# Autodesk Inventor assembly: POM_T5_16
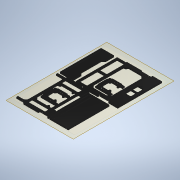
[picture p0: Inventor's stored thumbnail of the model, 180x180]
Saved by Autodesk Inventor 2020 (Build 240168000, 168)
## iProperties
Created: 2021-08-27
Part Number: POM_T5_16
Document SubType Name: Assembly
Designer: Masato
Author: Masato
## Documents named in this file (8)
- C:\Inventor\SUSTAINA-OP\Cam\POM_T5_16.iam
- C:\Inventor\SUSTAINA-OP\Cam\DisposableBoard.ipt
- C:\Inventor\SUSTAINA-OP\UpperBody\Cockpit\Cockpit_front_frame.ipt
- C:\Inventor\SUSTAINA-OP\UpperBody\Cockpit\Cockpit_carrier_board_frame.ipt
- C:\Inventor\SUSTAINA-OP\UpperBody\Cockpit\Cockpit_circuit_board_frame.ipt
- C:\Inventor\SUSTAINA-OP\UpperBody\Cockpit\Cockpit_battery_back_door.ipt
- C:\Inventor\SUSTAINA-OP\UpperBody\Cockpit\Cockpit_top_frame.ipt
- C:\Inventor\SUSTAINA-OP\UpperBody\Head\Camera_root_frame_e-CAM50_CUNX.ipt
## Components (8 placed, 7 different names)
1. DisposableBoard:1 — メイト:2, メイト:1, フラッシュ:1, フラッシュ:2, メイト:4, メイト:5, メイト:6, メイト:7, フラッシュ:3, フラッシュ:4, メイト:13, メイト:14, メイト:15
2. Cockpit_front_frame:1 — メイト:4, フラッシュ:5, メイト:9
3. Cockpit_carrier_board_frame:1 — メイト:5, フラッシュ:3, フラッシュ:4, フラッシュ:5, フラッシュ:6, メイト:8, メイト:9, メイト:10, メイト:11, メイト:16, メイト:17
4. Cockpit_circuit_board_frame:1 — メイト:7, メイト:10, メイト:11, メイト:12, フラッシュ:7, メイト:18, メイト:19
5. Cockpit_battery_back_door:1 — メイト:6, フラッシュ:6, メイト:8
6. Cockpit_top_frame:1 — メイト:12, メイト:13, フラッシュ:7
7. Camera_root_frame_e-CAM50_CUNX:1 — メイト:14, メイト:16, メイト:17
8. Camera_root_frame_e-CAM50_CUNX:2 — メイト:15, メイト:18, メイト:19
## Relationships (25: Mate 18, Flush 7)
- メイト:2 [Mate]: DisposableBoard:1
- メイト:1 [Mate]: DisposableBoard:1
- フラッシュ:1 [Flush]: DisposableBoard:1
- フラッシュ:2 [Flush]: DisposableBoard:1
- メイト:4 [Mate]: DisposableBoard:1 ↔ Cockpit_front_frame:1
- メイト:5 [Mate]: DisposableBoard:1 ↔ Cockpit_carrier_board_frame:1
- メイト:6 [Mate]: DisposableBoard:1 ↔ Cockpit_battery_back_door:1
- メイト:7 [Mate]: DisposableBoard:1 ↔ Cockpit_circuit_board_frame:1
- フラッシュ:3 [Flush] (2 mm): DisposableBoard:1 ↔ Cockpit_carrier_board_frame:1
- フラッシュ:4 [Flush] (2 mm): DisposableBoard:1 ↔ Cockpit_carrier_board_frame:1
- フラッシュ:5 [Flush]: Cockpit_front_frame:1 ↔ Cockpit_carrier_board_frame:1
- フラッシュ:6 [Flush]: Cockpit_carrier_board_frame:1 ↔ Cockpit_battery_back_door:1
- メイト:8 [Mate] (2.5 mm): Cockpit_carrier_board_frame:1 ↔ Cockpit_battery_back_door:1
- メイト:9 [Mate] (2.5 mm): Cockpit_front_frame:1 ↔ Cockpit_carrier_board_frame:1
- メイト:10 [Mate] (2.5 mm): Cockpit_carrier_board_frame:1 ↔ Cockpit_circuit_board_frame:1
- メイト:11 [Mate] (2.5 mm): Cockpit_carrier_board_frame:1 ↔ Cockpit_circuit_board_frame:1
- メイト:12 [Mate] (2.5 mm): Cockpit_circuit_board_frame:1 ↔ Cockpit_top_frame:1
- メイト:13 [Mate]: DisposableBoard:1 ↔ Cockpit_top_frame:1
- フラッシュ:7 [Flush]: Cockpit_circuit_board_frame:1 ↔ Cockpit_top_frame:1
- メイト:14 [Mate]: DisposableBoard:1 ↔ Camera_root_frame_e-CAM50_CUNX:1
- メイト:15 [Mate]: DisposableBoard:1 ↔ Camera_root_frame_e-CAM50_CUNX:2
- メイト:16 [Mate] (4 mm): Cockpit_carrier_board_frame:1 ↔ Camera_root_frame_e-CAM50_CUNX:1
- メイト:17 [Mate] (16.5 mm): Cockpit_carrier_board_frame:1 ↔ Camera_root_frame_e-CAM50_CUNX:1
- メイト:18 [Mate] (7 mm): Cockpit_circuit_board_frame:1 ↔ Camera_root_frame_e-CAM50_CUNX:2
- メイト:19 [Mate] (7.5 mm): Cockpit_circuit_board_frame:1 ↔ Camera_root_frame_e-CAM50_CUNX:2
